# Autodesk Inventor assembly: guide
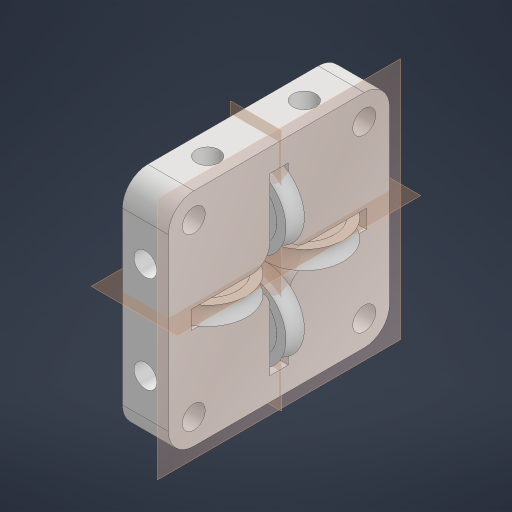
[picture p0: Inventor's stored thumbnail of the model, 512x512]
Saved by Autodesk Inventor 2024 (Build 280153000, 153)
## iProperties
Created: 2026-03-27
Part Number: guide
Document SubType Name: Assembly
Designer: schar
Author: schar
## Documents named in this file (3)
- C:\Users\schar\Desktop\FloatingFace\models\guide.iam
- C:\Users\schar\Desktop\FloatingFace\models\guidance_block.ipt
- C:\Users\schar\Desktop\FloatingFace\models\guide_bearing_assembly.iam
## Components (5 placed, 2 different names)
1. guidance_block:1 — Mate:1, Mate:2, Mate:3, Mate:4, Mate:5, Mate:6, Mate:7, Mate:8, Flush:1, Angle:1, Flush:3
2. guide_bearing_assembly:1 [sub-assembly] — Mate:1, Mate:2
3. guide_bearing_assembly:2 [sub-assembly] — Mate:7, Mate:8
4. guide_bearing_assembly:3 [sub-assembly] — Mate:3, Mate:4
5. guide_bearing_assembly:4 [sub-assembly] — Mate:5, Mate:6, Tangent:1
## Relationships (13: Mate 8, Flush 3, Angle 1, Tangent 1)
- Mate:1: guidance_block:1 ↔ guide_bearing_assembly:1
- Mate:2: guidance_block:1 ↔ guide_bearing_assembly:1
- Mate:3: guidance_block:1 ↔ guide_bearing_assembly:3
- Mate:4: guidance_block:1 ↔ guide_bearing_assembly:3
- Mate:5: guidance_block:1 ↔ guide_bearing_assembly:4
- Mate:6: guidance_block:1 ↔ guide_bearing_assembly:4
- Mate:7: guidance_block:1 ↔ guide_bearing_assembly:2
- Mate:8: guidance_block:1 ↔ guide_bearing_assembly:2
- Flush:1 (-24 mm): guidance_block:1
- Angle:1 (0 deg): guidance_block:1
- Tangent:1: guide_bearing_assembly:4
- Flush:2 (-1.172 mm)
- Flush:3: guidance_block:1
